# Autodesk Inventor assembly: Assembly_v1
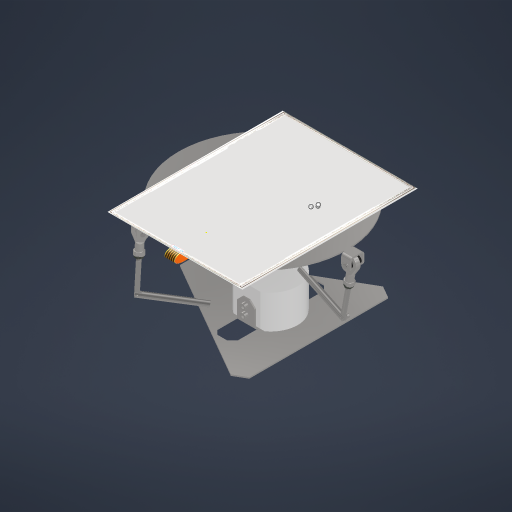
[picture p0: Inventor's stored thumbnail of the model, 512x512]
Saved by Autodesk Inventor 2023 (Build 270158000, 158)
## iProperties
Created: 2023-02-24
Part Number: Assembly_v1
Document SubType Name: Assembly
Designer: roota
Author: roota
## Documents named in this file (30)
- D:\GitHub\NTUST-Mechanical-Design\Ball stabilization mechanism\3D CAD files\Mechanical Part CAD files\Assemblies\Assembly_v1.iam
- D:\GitHub\NTUST-Mechanical-Design\Ball stabilization mechanism\3D CAD files\Mechanical Part CAD files\Static Mechanisms\BalancePlate.ipt
- D:\GitHub\NTUST-Mechanical-Design\Ball stabilization mechanism\3D CAD files\Mechanical Part CAD files\Static Mechanisms\BasePlate.ipt
- D:\GitHub\NTUST-Mechanical-Design\Ball stabilization mechanism\3D CAD files\Mechanical Part CAD files\Static Mechanisms\BaseSupport.ipt
- C:\Users\roota\Documents\Inventor\Content Center Files\R2023\en-US\JIS B 2804 E\_JIS B 2804 E - 5 - 6.ipt
- D:\GitHub\NTUST-Mechanical-Design\Ball stabilization mechanism\3D CAD files\Mechanical Part CAD files\Static Mechanisms\rod pin.ipt
- D:\GitHub\NTUST-Mechanical-Design\Ball stabilization mechanism\3D CAD files\Mechanical Part CAD files\Static Mechanisms\4mm spacer.ipt
- D:\GitHub\NTUST-Mechanical-Design\Ball stabilization mechanism\3D CAD files\Mechanical Part CAD files\Hardware Parts\SELF-LUBRIFICATING ROD END\Ball_6mm.ipt
- D:\GitHub\NTUST-Mechanical-Design\Ball stabilization mechanism\3D CAD files\Mechanical Part CAD files\Hardware Parts\SELF-LUBRIFICATING ROD END\End_6mm.ipt
- D:\GitHub\NTUST-Mechanical-Design\Ball stabilization mechanism\3D CAD files\Mechanical Part CAD files\Hardware Parts\M6x1_THREADED_ROD.ipt
- D:\GitHub\NTUST-Mechanical-Design\Ball stabilization mechanism\3D CAD files\Mechanical Part CAD files\Hardware Parts\5mm Bushing.ipt
- D:\GitHub\NTUST-Mechanical-Design\Ball stabilization mechanism\3D CAD files\Mechanical Part CAD files\Dynamic Mechanisms\Servo_Strut.ipt
- C:\Users\roota\Documents\Inventor\Content Center Files\R2023\en-US\ISO 4762(2)\ISO 4762 - M3 x 8ISO.ipt
- D:\GitHub\NTUST-Mechanical-Design\Ball stabilization mechanism\3D CAD files\Mechanical Part CAD files\Hardware Parts\12_1_INCH_TOUCHSCREEN\12inch Touchscreen.ipt
- C:\Users\roota\Documents\Inventor\Content Center Files\R2023\en-US\ISO 4036(2)\ISO 4036 - M6(2).ipt
- D:\GitHub\NTUST-Mechanical-Design\Ball stabilization mechanism\3D CAD files\Mechanical Part CAD files\Static Mechanisms\rod pin_CPY.ipt
- D:\GitHub\NTUST-Mechanical-Design\Ball stabilization mechanism\3D CAD files\Mechanical Part CAD files\Static Mechanisms\4mm spacer_CPY.ipt
- D:\GitHub\NTUST-Mechanical-Design\Ball stabilization mechanism\3D CAD files\Mechanical Part CAD files\Hardware Parts\SELF-LUBRIFICATING ROD END\Ball_6mm_CPY.ipt
- D:\GitHub\NTUST-Mechanical-Design\Ball stabilization mechanism\3D CAD files\Mechanical Part CAD files\Hardware Parts\SELF-LUBRIFICATING ROD END\End_6mm_CPY.ipt
- D:\GitHub\NTUST-Mechanical-Design\Ball stabilization mechanism\3D CAD files\Mechanical Part CAD files\Hardware Parts\M6x1_THREADED_ROD_CPY.ipt
- D:\GitHub\NTUST-Mechanical-Design\Ball stabilization mechanism\3D CAD files\Mechanical Part CAD files\Hardware Parts\5mm Bushing_CPY.ipt
- D:\GitHub\NTUST-Mechanical-Design\Ball stabilization mechanism\3D CAD files\Mechanical Part CAD files\Dynamic Mechanisms\Servo_Strut_CPY.ipt
- D:\GitHub\NTUST-Mechanical-Design\Ball stabilization mechanism\3D CAD files\Mechanical Part CAD files\Static Mechanisms\rod pin_CPY_CPY.ipt
- D:\GitHub\NTUST-Mechanical-Design\Ball stabilization mechanism\3D CAD files\Mechanical Part CAD files\Static Mechanisms\4mm spacer_CPY_CPY.ipt
- D:\GitHub\NTUST-Mechanical-Design\Ball stabilization mechanism\3D CAD files\Mechanical Part CAD files\Hardware Parts\SELF-LUBRIFICATING ROD END\Ball_6mm_CPY_CPY.ipt
- D:\GitHub\NTUST-Mechanical-Design\Ball stabilization mechanism\3D CAD files\Mechanical Part CAD files\Hardware Parts\SELF-LUBRIFICATING ROD END\End_6mm_CPY_CPY.ipt
- D:\GitHub\NTUST-Mechanical-Design\Ball stabilization mechanism\3D CAD files\Mechanical Part CAD files\Hardware Parts\M6x1_THREADED_ROD_CPY_CPY.ipt
- D:\GitHub\NTUST-Mechanical-Design\Ball stabilization mechanism\3D CAD files\Mechanical Part CAD files\Hardware Parts\5mm Bushing_CPY_CPY.ipt
- D:\GitHub\NTUST-Mechanical-Design\Ball stabilization mechanism\3D CAD files\Mechanical Part CAD files\Dynamic Mechanisms\Servo_Strut_CPY_CPY.ipt
- C:\Users\roota\Documents\Inventor\Content Center Files\R2023\en-US\ISO 4762(2)\ISO 4762 - M5 x 8ISO.ipt
## Components (44 placed, 29 different names)
1. BalancePlate:1 — Mate:6, Mate:9, Mate:10, Mate:11, Mate:12, Mate:60, Mate:61, Mate:62, Mate:63, Mate:64, Mate:65, Mate:66, Mate:67, Mate:68, Flush:1, Flush:2
2. BasePlate:1 — Mate:1, Mate:2, Mate:3, Insert:4, Insert:5, Insert:6, Insert:7
3. BaseSupport:1 — Mate:1, Mate:2, Mate:3
4. JIS B 2804 E 5:5 — Mate:5, Mate:8, Mate:10
5. JIS B 2804 E 5:6 — Mate:4, Mate:7
6. rod pin:3 — Mate:4, Mate:5, Mate:6, Mate:7, Mate:8, Mate:9, Mate:13, Mate:14, Mate:15
7. 4mm spacer:1 — Mate:12, Mate:13
8. 4mm spacer:2 — Mate:11, Mate:14, Mate:16
9. Ball_6mm:1 — Mate:15, Mate:16, Mate:17
10. End_6mm:1 — Mate:17, Mate:18, Mate:19, Angle:1, Insert:1
11. M6x1_THREADED_ROD:1 — Mate:18, Mate:19, Mate:20, Mate:23, Angle:1
12. 5mm Bushing:1 — Mate:20, Mate:21, Mate:22, Mate:24
13. Servo_Strut:1 — Mate:21, Mate:22, Mate:23, Mate:25
14. ISO 4762 M3 x 8:1 — Mate:24, Mate:25
15. ISO 4036 M6:1 — Insert:1
16. 12inch Touchscreen:1 — Mate:68, Flush:1, Flush:2
17. JIS B 2804 E 5:7 — Mate:26, Mate:28
18. JIS B 2804 E 5:8 — Mate:27, Mate:29, Mate:62
19. rod pin_CPY:1 — Mate:26, Mate:27, Mate:28, Mate:29, Mate:30, Mate:31, Mate:33
20. 4mm spacer_CPY:1 — Mate:30, Mate:60, Mate:61
21. 4mm spacer_CPY:2 — Mate:31, Mate:32, Mate:63
22. Ball_6mm_CPY:1 — Mate:32, Mate:33, Mate:34
23. End_6mm_CPY:1 — Mate:34, Angle:2, Mate:35, Mate:36, Insert:2
24. M6x1_THREADED_ROD_CPY:1 — Angle:2, Mate:35, Mate:36, Mate:37, Mate:38
25. 5mm Bushing_CPY:1 — Mate:37, Mate:39, Mate:40, Mate:42
26. Servo_Strut_CPY:1 — Mate:38, Mate:39, Mate:40, Mate:41
27. ISO 4762 M3 x 8:2 — Mate:41, Mate:42
28. ISO 4036 M6:2 — Insert:2
29. JIS B 2804 E 5:9 — Mate:44, Mate:46
30. JIS B 2804 E 5:10 — Mate:43, Mate:45, Mate:67
31. rod pin_CPY_CPY:1 — Mate:43, Mate:44, Mate:45, Mate:46, Mate:47, Mate:48, Mate:49
32. 4mm spacer_CPY_CPY:1 — Mate:47, Mate:66
33. 4mm spacer_CPY_CPY:2 — Mate:48, Mate:50, Mate:64, Mate:65
34. Ball_6mm_CPY_CPY:1 — Mate:49, Mate:50, Mate:51
35. End_6mm_CPY_CPY:1 — Mate:51, Mate:52, Mate:53, Angle:3, Insert:3
36. M6x1_THREADED_ROD_CPY_CPY:1 — Mate:52, Mate:53, Angle:3, Mate:54, Mate:57
37. 5mm Bushing_CPY_CPY:1 — Mate:54, Mate:55, Mate:56, Mate:58
38. Servo_Strut_CPY_CPY:1 — Mate:55, Mate:56, Mate:57, Mate:59
39. ISO 4762 M3 x 8:3 — Mate:58, Mate:59
40. ISO 4036 M6:3 — Insert:3
41. ISO 4762 M5 x 8:1 — Insert:4
42. ISO 4762 M5 x 8:2 — Insert:5
43. ISO 4762 M5 x 8:3 — Insert:6
44. ISO 4762 M5 x 8:4 — Insert:7
## Relationships (80: Mate 68, Insert 7, Angle 3, Flush 2)
- Mate:1: BasePlate:1 ↔ BaseSupport:1
- Mate:2: BasePlate:1 ↔ BaseSupport:1
- Mate:3: BasePlate:1 ↔ BaseSupport:1
- Mate:4: JIS B 2804 E 5:6 ↔ rod pin:3
- Mate:5: JIS B 2804 E 5:5 ↔ rod pin:3
- Mate:6: BalancePlate:1 ↔ rod pin:3
- Mate:7: JIS B 2804 E 5:6 ↔ rod pin:3
- Mate:8: JIS B 2804 E 5:5 ↔ rod pin:3
- Mate:9: BalancePlate:1 ↔ rod pin:3
- Mate:10: BalancePlate:1 ↔ JIS B 2804 E 5:5
- Mate:11: BalancePlate:1 ↔ 4mm spacer:2
- Mate:12: BalancePlate:1 ↔ 4mm spacer:1
- Mate:13: rod pin:3 ↔ 4mm spacer:1
- Mate:14: rod pin:3 ↔ 4mm spacer:2
- Mate:15: rod pin:3 ↔ Ball_6mm:1
- Mate:16: 4mm spacer:2 ↔ Ball_6mm:1
- Mate:17: Ball_6mm:1 ↔ End_6mm:1
- Mate:18: End_6mm:1 ↔ M6x1_THREADED_ROD:1
- Mate:19 (-8 mm): End_6mm:1 ↔ M6x1_THREADED_ROD:1
- Mate:20: M6x1_THREADED_ROD:1 ↔ 5mm Bushing:1
- Mate:21: 5mm Bushing:1 ↔ Servo_Strut:1
- Mate:22: 5mm Bushing:1 ↔ Servo_Strut:1
- Mate:23: M6x1_THREADED_ROD:1 ↔ Servo_Strut:1
- Angle:1 (0 deg): End_6mm:1 ↔ M6x1_THREADED_ROD:1
- Mate:24: 5mm Bushing:1 ↔ ISO 4762 M3 x 8:1
- Mate:25: Servo_Strut:1 ↔ ISO 4762 M3 x 8:1
- Insert:1: End_6mm:1 ↔ ISO 4036 M6:1
- Mate:26: JIS B 2804 E 5:7 ↔ rod pin_CPY:1
- Mate:27: JIS B 2804 E 5:8 ↔ rod pin_CPY:1
- Mate:28: JIS B 2804 E 5:7 ↔ rod pin_CPY:1
- Mate:29: JIS B 2804 E 5:8 ↔ rod pin_CPY:1
- Mate:30: rod pin_CPY:1 ↔ 4mm spacer_CPY:1
- Mate:31: rod pin_CPY:1 ↔ 4mm spacer_CPY:2
- Mate:32: 4mm spacer_CPY:2 ↔ Ball_6mm_CPY:1
- Mate:33: rod pin_CPY:1 ↔ Ball_6mm_CPY:1
- Mate:34: Ball_6mm_CPY:1 ↔ End_6mm_CPY:1
- Angle:2 (0 deg): End_6mm_CPY:1 ↔ M6x1_THREADED_ROD_CPY:1
- Mate:35 (-8 mm): End_6mm_CPY:1 ↔ M6x1_THREADED_ROD_CPY:1
- Mate:36: End_6mm_CPY:1 ↔ M6x1_THREADED_ROD_CPY:1
- Mate:37: M6x1_THREADED_ROD_CPY:1 ↔ 5mm Bushing_CPY:1
- Mate:38: M6x1_THREADED_ROD_CPY:1 ↔ Servo_Strut_CPY:1
- Mate:39: 5mm Bushing_CPY:1 ↔ Servo_Strut_CPY:1
- Mate:40: 5mm Bushing_CPY:1 ↔ Servo_Strut_CPY:1
- Mate:41: Servo_Strut_CPY:1 ↔ ISO 4762 M3 x 8:2
- Mate:42: 5mm Bushing_CPY:1 ↔ ISO 4762 M3 x 8:2
- Insert:2: End_6mm_CPY:1 ↔ ISO 4036 M6:2
- Mate:43: JIS B 2804 E 5:10 ↔ rod pin_CPY_CPY:1
- Mate:44: JIS B 2804 E 5:9 ↔ rod pin_CPY_CPY:1
- Mate:45: JIS B 2804 E 5:10 ↔ rod pin_CPY_CPY:1
- Mate:46: JIS B 2804 E 5:9 ↔ rod pin_CPY_CPY:1
- Mate:47: rod pin_CPY_CPY:1 ↔ 4mm spacer_CPY_CPY:1
- Mate:48: rod pin_CPY_CPY:1 ↔ 4mm spacer_CPY_CPY:2
- Mate:49: rod pin_CPY_CPY:1 ↔ Ball_6mm_CPY_CPY:1
- Mate:50: 4mm spacer_CPY_CPY:2 ↔ Ball_6mm_CPY_CPY:1
- Mate:51: Ball_6mm_CPY_CPY:1 ↔ End_6mm_CPY_CPY:1
- Mate:52: End_6mm_CPY_CPY:1 ↔ M6x1_THREADED_ROD_CPY_CPY:1
- Mate:53 (-8 mm): End_6mm_CPY_CPY:1 ↔ M6x1_THREADED_ROD_CPY_CPY:1
- Angle:3 (0 deg): End_6mm_CPY_CPY:1 ↔ M6x1_THREADED_ROD_CPY_CPY:1
- Mate:54: M6x1_THREADED_ROD_CPY_CPY:1 ↔ 5mm Bushing_CPY_CPY:1
- Mate:55: 5mm Bushing_CPY_CPY:1 ↔ Servo_Strut_CPY_CPY:1
- Mate:56: 5mm Bushing_CPY_CPY:1 ↔ Servo_Strut_CPY_CPY:1
- Mate:57: M6x1_THREADED_ROD_CPY_CPY:1 ↔ Servo_Strut_CPY_CPY:1
- Mate:58: 5mm Bushing_CPY_CPY:1 ↔ ISO 4762 M3 x 8:3
- Mate:59: Servo_Strut_CPY_CPY:1 ↔ ISO 4762 M3 x 8:3
- Insert:3: End_6mm_CPY_CPY:1 ↔ ISO 4036 M6:3
- Mate:60: BalancePlate:1 ↔ 4mm spacer_CPY:1
- Mate:61: BalancePlate:1 ↔ 4mm spacer_CPY:1
- Mate:62: BalancePlate:1 ↔ JIS B 2804 E 5:8
- Mate:63: BalancePlate:1 ↔ 4mm spacer_CPY:2
- Mate:64: BalancePlate:1 ↔ 4mm spacer_CPY_CPY:2
- Mate:65: BalancePlate:1 ↔ 4mm spacer_CPY_CPY:2
- Mate:66: BalancePlate:1 ↔ 4mm spacer_CPY_CPY:1
- Mate:67: BalancePlate:1 ↔ JIS B 2804 E 5:10
- Insert:4: BasePlate:1 ↔ ISO 4762 M5 x 8:1
- Insert:5: BasePlate:1 ↔ ISO 4762 M5 x 8:2
- Insert:6: BasePlate:1 ↔ ISO 4762 M5 x 8:3
- Insert:7: BasePlate:1 ↔ ISO 4762 M5 x 8:4
- Mate:68: BalancePlate:1 ↔ 12inch Touchscreen:1
- Flush:1 (-40 mm): BalancePlate:1 ↔ 12inch Touchscreen:1
- Flush:2 (120 mm): BalancePlate:1 ↔ 12inch Touchscreen:1
